# Autodesk Inventor assembly: 回転軸フレーム
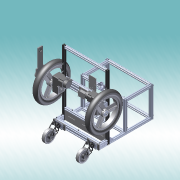
[picture p0: Inventor's stored thumbnail of the model, 180x180]
Saved by Autodesk Inventor 2015 (Build 190159000, 159)
## iProperties
Created: 2016-02-29
Part Number: 回転軸フレーム
Document SubType Name: Assembly
Designer: buzztaka
Author: buzztaka
## Documents named in this file (50)
- C:\Users\buzztaka\Documents\tukuba\i-cart-middle_3d-model\計測輪アセンブル\回転軸フレーム (ベアリングホルダ使用).iam
- C:\Users\buzztaka\Documents\tukuba\i-cart-middle_3d-model\計測輪アセンブル\wheel_12inch.ipt
- C:\Users\buzztaka\Documents\tukuba\i-cart-middle_3d-model\計測輪アセンブル\wheel-cap.ipt
- C:\Users\buzztaka\Documents\tukuba\i-cart-middle_3d-model\計測輪アセンブル\wheel-hub.ipt
- C:\Users\buzztaka\Documents\tukuba\i-cart-middle_3d-model\計測輪アセンブル\hblfsn5.ipt
- C:\Users\buzztaka\Documents\tukuba\i-cart-middle_3d-model\計測輪アセンブル\hblfsnf5.ipt
- C:\Users\buzztaka\Documents\tukuba\i-cart-middle_3d-model\計測輪アセンブル\HBLFSSW5.ipt
- C:\Users\buzztaka\Documents\tukuba\i-cart-middle_3d-model\計測輪アセンブル\hntaj5_5.ipt
- C:\Users\buzztaka\Documents\tukuba\i-cart-middle_3d-model\計測輪アセンブル\MTi-30.ipt
- C:\Users\buzztaka\Documents\tukuba\i-cart-middle_3d-model\計測輪アセンブル\HFSB5-2020-550-LCH-RWV-AH30-BH240-CH280-DH442-EH462.ipt
- C:\Users\buzztaka\Documents\tukuba\i-cart-middle_3d-model\計測輪アセンブル\HFSB5-2020-550-LCH-RWV-AH30-BH60-CH85-DH240-EH280-AP442.ipt
- C:\Users\buzztaka\Documents\tukuba\i-cart-middle_3d-model\計測輪アセンブル\C-SFL6901ZZ.ipt
- C:\Users\buzztaka\Documents\tukuba\i-cart-middle_3d-model\計測輪アセンブル\タイヤアーム.ipt
- C:\Users\buzztaka\Documents\tukuba\i-cart-middle_3d-model\計測輪アセンブル\meh-30-pエンコーダ.ipt
- C:\Users\buzztaka\Documents\tukuba\i-cart-middle_3d-model\計測輪アセンブル\スプリングフランジ用ワッシャー（座金）.ipt
- C:\Users\buzztaka\Documents\tukuba\i-cart-middle_3d-model\計測輪アセンブル\スプリングフランジ0.1mm.ipt
- C:\Users\buzztaka\Documents\tukuba\i-cart-middle_3d-model\計測輪アセンブル\ힼ�ힼ�ힼ�ힼ�.ipt
- C:\Users\buzztaka\Documents\tukuba\i-cart-middle_3d-model\計測輪アセンブル\ힼ�ힼ�ힼ�ힼ�ힼ�-L1.ipt
- C:\Users\buzztaka\Documents\tukuba\i-cart-middle_3d-model\計測輪アセンブル\ힼ�ힼ�ힼ�ힼ�ힼ�-L2.ipt
- C:\Users\buzztaka\Documents\tukuba\i-cart-middle_3d-model\計測輪アセンブル\ힼ�ힼ�ힼ�ힼ�ힼ�-ힽ�ힽ�.ipt
- C:\Users\buzztaka\Documents\tukuba\i-cart-middle_3d-model\計測輪アセンブル\ힼ�ힼ�ힼ�ힼ�ힼ�-ힼ�ힽ�ힽ�.ipt
- C:\Users\buzztaka\Documents\tukuba\i-cart-middle_3d-model\計測輪アセンブル\ힼ�ힼ�ힼ�ힼ�-ힼ�ힽ�ힽ�Lힼ�ힼ�ힼ�ힼ�ힼ�.ipt
- C:\Users\buzztaka\Documents\tukuba\i-cart-middle_3d-model\計測輪アセンブル\ힼ�ힼ�ힼ�ힼ�ힼ�-ힼ�ힼ�ힼ�ힼ�ힼ�ힽ�ힼ�ힼ�ힽ�.ipt
- C:\Users\buzztaka\Documents\tukuba\i-cart-middle_3d-model\計測輪アセンブル\ힼ�ힼ�ힼ�ힼ�(ힽ�ힽ�).ipt
- C:\Users\buzztaka\Documents\tukuba\i-cart-middle_3d-model\計測輪アセンブル\ힼ�ힼ�ힼ�ힼ�ힼ�ힼ�ힼ�-2020-L2.ipt
- C:\Users\buzztaka\Documents\tukuba\i-cart-middle_3d-model\計測輪アセンブル\ힼ�ힼ�ힼ�ힼ�ힼ�ힼ�ힼ�-2040-L2.ipt
- C:\Users\buzztaka\Documents\tukuba\i-cart-middle_3d-model\計測輪アセンブル\ힼ�ힼ�ힼ�ힼ�ힼ�ힼ�ힼ�-2060-L2.ipt
- C:\Users\buzztaka\Documents\tukuba\i-cart-middle_3d-model\計測輪アセンブル\ힼ�ힼ�ힼ�ힼ�ힼ�ힼ�ힼ�-2040-L3.ipt
- C:\Users\buzztaka\Documents\tukuba\i-cart-middle_3d-model\計測輪アセンブル\ힼ�ힼ�ힼ�ힼ�ힼ�ힼ�ힼ�-2020-L4.ipt
- C:\Users\buzztaka\Documents\tukuba\i-cart-middle_3d-model\計測輪アセンブル\ힼ�ힼ�ힼ�ힼ�ힼ�ힼ�ힼ�-2020-L5.ipt
- C:\Users\buzztaka\Documents\tukuba\i-cart-middle_3d-model\計測輪アセンブル\ힼ�ힼ�ힼ�ힼ�ힼ�ힼ�ힼ�-2020-L6.ipt
- C:\Users\buzztaka\Documents\tukuba\i-cart-middle_3d-model\計測輪アセンブル\ힼ�ힼ�ힼ�ힼ�ힼ�ힼ�ힼ�-2020-L7.ipt
- C:\Users\buzztaka\Documents\tukuba\i-cart-middle_3d-model\計測輪アセンブル\ힼ�ힼ�ힼ�ힼ�ힼ�ힼ�ힼ�-ힽ�ힽ�ힽ�ힼ�ힼ�ힼ�ힼ�ힼ�ힼ�.ipt
- C:\Users\buzztaka\Documents\tukuba\i-cart-middle_3d-model\計測輪アセンブル\ힼ�ힼ�ힼ�ힼ�ힼ�ힼ�ힼ�-ힼ�ힼ�ힼ�-M5.ipt
- C:\Users\buzztaka\Documents\tukuba\i-cart-middle_3d-model\計測輪アセンブル\ힼ�ힼ�ힼ�ힼ�ힼ�ힼ�ힼ�-ힽ�ힼ�ힽ�ힼ�ힼ�.ipt
- C:\Users\buzztaka\Documents\tukuba\i-cart-middle_3d-model\計測輪アセンブル\URG_ힼ�ힽ�ힽ�ힼ�ힼ�ힼ�ힽ�.ipt
- C:\Users\buzztaka\Documents\tukuba\i-cart-middle_3d-model\計測輪アセンブル\imu_ힼ�ힼ�ힼ�ힼ�.ipt
- C:\Users\buzztaka\Documents\tukuba\i-cart-middle_3d-model\計測輪アセンブル\ힽ�ힼ�ힼ�ힼ�ힼ�ힽ�.ipt
- C:\Users\buzztaka\Documents\tukuba\i-cart-middle_3d-model\計測輪アセンブル\M3ힽ�ힼ�ힼ�ힼ�ힼ�ힼ�ힼ�.ipt
- C:\Users\buzztaka\Documents\tukuba\i-cart-middle_3d-model\計測輪アセンブル\ힼ�ힼ�ힼ�-M5.ipt
- C:\Users\buzztaka\Documents\tukuba\i-cart-middle_3d-model\計測輪アセンブル\ힼ�ힼ�-Cap-M5-12.ipt
- C:\Users\buzztaka\Documents\tukuba\i-cart-middle_3d-model\計測輪アセンブル\ힼ�ힼ�-Cap-M5-10.ipt
- C:\Users\buzztaka\Documents\tukuba\i-cart-middle_3d-model\計測輪アセンブル\ힼ�ힼ�-Cap-M5-8.ipt
- C:\Users\buzztaka\Documents\tukuba\i-cart-middle_3d-model\計測輪アセンブル\ힼ�ힼ�-ힼ�ힼ�-M5.ipt
- C:\Users\buzztaka\Documents\tukuba\i-cart-middle_3d-model\計測輪アセンブル\ힼ�ힼ�-ힼ�ힼ�-M3.ipt
- C:\Users\buzztaka\Documents\tukuba\i-cart-middle_3d-model\計測輪アセンブル\ힼ�ힼ�-Cap-M3-6.ipt
- C:\Users\buzztaka\Documents\tukuba\i-cart-middle_3d-model\計測輪アセンブル\ힼ�ힼ�-Cap-M5-60.ipt
- C:\Users\buzztaka\Documents\tukuba\i-cart-middle_3d-model\計測輪アセンブル\ힼ�ힼ�-Cap-M6-10.ipt
- C:\Users\buzztaka\Documents\tukuba\i-cart-middle_3d-model\計測輪アセンブル\ힼ�ힼ�-ힼ�ힼ�ힼ�-M3-16.ipt
- C:\Users\buzztaka\Documents\tukuba\i-cart-middle_3d-model\計測輪アセンブル\ힼ�ힼ�ힽ�-M5.ipt
## Components (52 placed, 15 different names)
1. wheel_12inch
2. wheel-cap
3. wheel-hub
4. hblfsn5
5. hblfsnf5:1
6. hblfsnf5:2
7. HBLFSSW5
8. hntaj5_5
9. hntaj5_5:1
10. hntaj5_5:2
11. hntaj5_5:3
12. hntaj5_5:4
13. hntaj5_5:5
14. hntaj5_5:6
15. hntaj5_5:12
16. hntaj5_5:16
17. hntaj5_5:17
18. hntaj5_5:18
19. hntaj5_5:19
20. hntaj5_5:20
21. hntaj5_5:21
22. hntaj5_5:22
23. hntaj5_5:23
24. hntaj5_5:24
25. hntaj5_5:25
26. wheel_12inch:1
27. wheel-cap:1
28. wheel-hub:1
29. MTi-30
30. hblfsn5:1
31. hblfsnf5:3
32. hntaj5_5:26
33. hntaj5_5:27
34. hntaj5_5:28
35. hntaj5_5:35
36. hntaj5_5:36
37. hntaj5_5:37
38. hntaj5_5:38
39. hntaj5_5:39
40. hntaj5_5:40
41. hntaj5_5:41
42. hntaj5_5:42
43. HFSB5-2020-550-LCH-RWV-AH30-BH240-CH280-DH442-EH462:2 — 挿入:3, 挿入:4
44. HFSB5-2020-550-LCH-RWV-AH30-BH60-CH85-DH240-EH280-AP442:1
45. C-SFL6901ZZ:4 — 挿入:40
46. タイヤアーム:1 — 挿入:40, 挿入:42, 挿入:48, 挿入:49
47. C-SFL6901ZZ:5 — 挿入:42
48. meh-30-pエンコーダ:1
49. スプリングフランジ用ワッシャー（座金）:1
50. スプリングフランジ用ワッシャー（座金）:2
51. スプリングフランジ用ワッシャー（座金）:3
52. スプリングフランジ0.1mm:1 — 挿入:48, 挿入:49
## Relationships (13: Insert 13)
- 挿入:3 [Insert]: HFSB5-2020-550-LCH-RWV-AH30-BH240-CH280-DH442-EH462:2
- 挿入:4 [Insert]: HFSB5-2020-550-LCH-RWV-AH30-BH240-CH280-DH442-EH462:2
- [Insert]: HFSB5-2020-550-LCH-RWV-AH30-BH60-CH85-DH240-EH280-AP442:1
- [Insert]: HFSB5-2020-550-LCH-RWV-AH30-BH60-CH85-DH240-EH280-AP442:1
- 挿入:40 [Insert]: C-SFL6901ZZ:4 ↔ タイヤアーム:1
- 挿入:42 [Insert]: タイヤアーム:1 ↔ C-SFL6901ZZ:5
- [Insert]: meh-30-pエンコーダ:1 ↔ スプリングフランジ用ワッシャー（座金）:2
- [Insert]: meh-30-pエンコーダ:1 ↔ スプリングフランジ用ワッシャー（座金）:1
- [Insert]: meh-30-pエンコーダ:1 ↔ スプリングフランジ用ワッシャー（座金）:3
- [Insert]: スプリングフランジ用ワッシャー（座金）:2 ↔ スプリングフランジ0.1mm:1
- [Insert]: スプリングフランジ用ワッシャー（座金）:3 ↔ スプリングフランジ0.1mm:1
- 挿入:48 [Insert]: タイヤアーム:1 ↔ スプリングフランジ0.1mm:1
- 挿入:49 [Insert]: タイヤアーム:1 ↔ スプリングフランジ0.1mm:1
